# Autodesk Inventor assembly: 膝_6_1
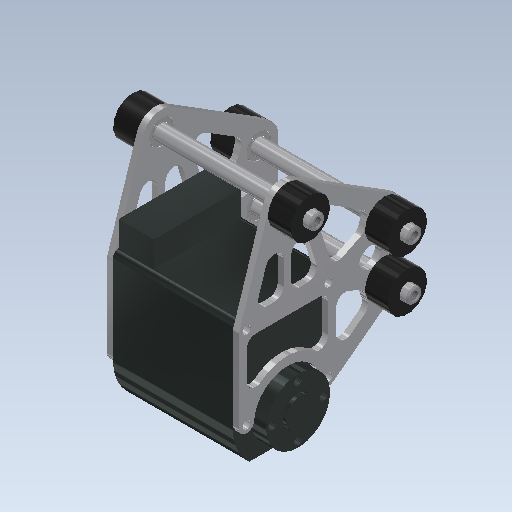
[picture p0: Inventor's stored thumbnail of the model, 512x512]
Saved by Autodesk Inventor 2020 (Build 240168000, 168)
## iProperties
Created: 2016-08-23
Part Number: 膝_6_1
Material: 一般
Document SubType Name: Assembly
Designer: hiro
Mass: 259.679 g
Surface Area: 513.454 cm^2
Volume: 137.54 cm^3
Density: 1.88802 g/cm^3
Author: hiro
## Documents named in this file (7)
- C:\Inventor\OpenPlatform_ver3_0\下半身_160823\膝\膝_6_1.iam
- C:\Inventor\OpenPlatform_ver3_0\既製品\B3M11xx.ipt
- C:\Inventor\OpenPlatform_ver3_0\下半身_160823\膝\膝_メインフレーム.ipt
- C:\Inventor\OpenPlatform_ver3_0\既製品\SETF5-63_5-M3-N3.ipt
- C:\Inventor\OpenPlatform_ver3_0\既製品\NSK_RB_MF85ZZ\MF85ZZ.iam
- C:\Inventor\OpenPlatform_ver3_0\既製品\free_horn.ipt
- C:\Inventor\OpenPlatform_ver3_0\下半身\リンク\スペーサ\膝_同軸_スペーサ_1_5.ipt
## Components (19 placed, 6 different names)
1. B3M11xx:2 — 挿入:92, 挿入:96, 挿入:97, 挿入:98, 挿入:99
2. 膝_メインフレーム:1 — 挿入:80, 挿入:81, 挿入:82, 挿入:98, 挿入:99
3. 膝_メインフレーム:2 — 挿入:77, 挿入:78, 挿入:79, 挿入:96, 挿入:97
4. SETF5-63_5-M3-N3:1 — 挿入:103
5. MF85ZZ:1 [sub-assembly] — 挿入:80, 挿入:93
6. MF85ZZ:2 [sub-assembly] — 挿入:82, 挿入:95
7. MF85ZZ:3 [sub-assembly] — 挿入:81, 挿入:94
8. MF85ZZ:4 [sub-assembly] — 挿入:77, 挿入:102
9. MF85ZZ:5 [sub-assembly] — 挿入:78, 挿入:101
10. MF85ZZ:6 [sub-assembly] — 挿入:79, 挿入:100
11. SETF5-63_5-M3-N3:2 — 挿入:105
12. SETF5-63_5-M3-N3:3 — 挿入:104
13. free_horn:1 — 挿入:92
14. 膝_同軸_スペーサ_1_5:1 — 挿入:95, 挿入:105
15. 膝_同軸_スペーサ_1_5:2 — 挿入:94, 挿入:104
16. 膝_同軸_スペーサ_1_5:3 — 挿入:93, 挿入:103
17. 膝_同軸_スペーサ_1_5:4 — 挿入:100
18. 膝_同軸_スペーサ_1_5:5 — 挿入:101
19. 膝_同軸_スペーサ_1_5:6 — 挿入:102
## Relationships (20: Insert 20)
- 挿入:77 [Insert]: 膝_メインフレーム:2 ↔ MF85ZZ:4
- 挿入:78 [Insert]: 膝_メインフレーム:2 ↔ MF85ZZ:5
- 挿入:79 [Insert]: 膝_メインフレーム:2 ↔ MF85ZZ:6
- 挿入:80 [Insert]: 膝_メインフレーム:1 ↔ MF85ZZ:1
- 挿入:81 [Insert]: 膝_メインフレーム:1 ↔ MF85ZZ:3
- 挿入:82 [Insert]: 膝_メインフレーム:1 ↔ MF85ZZ:2
- 挿入:92 [Insert]: B3M11xx:2 ↔ free_horn:1
- 挿入:93 [Insert]: MF85ZZ:1 ↔ 膝_同軸_スペーサ_1_5:3
- 挿入:94 [Insert]: MF85ZZ:3 ↔ 膝_同軸_スペーサ_1_5:2
- 挿入:95 [Insert]: MF85ZZ:2 ↔ 膝_同軸_スペーサ_1_5:1
- 挿入:96 [Insert]: B3M11xx:2 ↔ 膝_メインフレーム:2
- 挿入:97 [Insert]: B3M11xx:2 ↔ 膝_メインフレーム:2
- 挿入:98 [Insert]: B3M11xx:2 ↔ 膝_メインフレーム:1
- 挿入:99 [Insert]: B3M11xx:2 ↔ 膝_メインフレーム:1
- 挿入:100 [Insert]: MF85ZZ:6 ↔ 膝_同軸_スペーサ_1_5:4
- 挿入:101 [Insert]: MF85ZZ:5 ↔ 膝_同軸_スペーサ_1_5:5
- 挿入:102 [Insert]: MF85ZZ:4 ↔ 膝_同軸_スペーサ_1_5:6
- 挿入:103 [Insert] (-2.5 mm): SETF5-63_5-M3-N3:1 ↔ 膝_同軸_スペーサ_1_5:3
- 挿入:104 [Insert] (-2.5 mm): SETF5-63_5-M3-N3:3 ↔ 膝_同軸_スペーサ_1_5:2
- 挿入:105 [Insert] (-2.5 mm): SETF5-63_5-M3-N3:2 ↔ 膝_同軸_スペーサ_1_5:1
